# Autodesk Inventor assembly: Eje delantero _1_
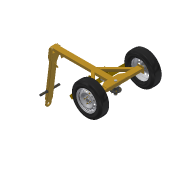
[picture p0: Inventor's stored thumbnail of the model, 180x180]
Saved by Autodesk Inventor 2019 (Build 230136000, 136)
## iProperties
Created: 2020-02-06
Part Number: Eje delantero _1_
Document SubType Name: Assembly
Designer: Juan Carlos Botero
Author: Juan Carlos Botero
## Documents named in this file (26)
- D:\Drives\OneDrive\Carlos_2\02 TRABAJOS\MULTIPLO\Conveyor\ENSAMBLE\Eje delantero _1_.iam
- D:\Drives\OneDrive\Carlos_2\02 TRABAJOS\MULTIPLO\Conveyor\ENSAMBLE\Seguro de tiro.ipt
- D:\Drives\OneDrive\Carlos_2\02 TRABAJOS\MULTIPLO\Conveyor\ENSAMBLE\Lamina bocin rueda.ipt
- D:\Drives\OneDrive\Carlos_2\02 TRABAJOS\MULTIPLO\Conveyor\ENSAMBLE\Lamina refuerzo eje quinta rueda.ipt
- D:\Drives\OneDrive\Carlos_2\02 TRABAJOS\MULTIPLO\Conveyor\ENSAMBLE\Lamina refuerzo tiro.ipt
- D:\Drives\OneDrive\Carlos_2\02 TRABAJOS\MULTIPLO\Conveyor\ENSAMBLE\Perfil tiro.ipt
- D:\Drives\OneDrive\Carlos_2\02 TRABAJOS\MULTIPLO\Conveyor\ENSAMBLE\Espaciador de nylon.ipt
- D:\Drives\OneDrive\Carlos_2\02 TRABAJOS\MULTIPLO\Conveyor\ENSAMBLE\Arandela de nylon (1).ipt
- D:\Drives\OneDrive\Carlos_2\02 TRABAJOS\MULTIPLO\Conveyor\ENSAMBLE\Refuerzo diagonal tiro (1).ipt
- D:\Drives\OneDrive\Carlos_2\02 TRABAJOS\MULTIPLO\Conveyor\ENSAMBLE\Barra quinta rueda.ipt
- D:\Drives\OneDrive\Carlos_2\02 TRABAJOS\MULTIPLO\Conveyor\ENSAMBLE\Lamina pivote seguro tiro.ipt
- D:\Drives\OneDrive\Carlos_2\02 TRABAJOS\MULTIPLO\Conveyor\ENSAMBLE\Tapa perfiles tiro.ipt
- D:\Drives\OneDrive\Carlos_2\02 TRABAJOS\MULTIPLO\Conveyor\ENSAMBLE\Rin 13_.ipt
- D:\Drives\OneDrive\Carlos_2\02 TRABAJOS\MULTIPLO\Conveyor\ENSAMBLE\70 R13.ipt
- D:\Drives\OneDrive\Carlos_2\02 TRABAJOS\MULTIPLO\Conveyor\ENSAMBLE\Bocin llantas _2_.iam
- D:\Drives\OneDrive\Carlos_2\02 TRABAJOS\MULTIPLO\Conveyor\ENSAMBLE\Bocin eje quinta rueda _1_.iam
- D:\Drives\OneDrive\Carlos_2\02 TRABAJOS\MULTIPLO\Conveyor\ENSAMBLE\Bocin llantas _1_.iam
- D:\Drives\OneDrive\Carlos_2\02 TRABAJOS\MULTIPLO\Conveyor\ENSAMBLE\Barra freno.ipt
- D:\Drives\OneDrive\Carlos_2\02 TRABAJOS\MULTIPLO\Conveyor\ENSAMBLE\Soporte freno.ipt
- D:\Drives\OneDrive\Carlos_2\02 TRABAJOS\MULTIPLO\Conveyor\ENSAMBLE\Soporte resorte freno.ipt
- D:\Drives\OneDrive\Carlos_2\02 TRABAJOS\MULTIPLO\Conveyor\ENSAMBLE\Eje delantero _1_\Design Accelerator\Extension Spring2.iam
- D:\Drives\OneDrive\Carlos_2\02 TRABAJOS\MULTIPLO\Conveyor\ENSAMBLE\Solid1.ipt
- D:\Drives\OneDrive\Carlos_2\02 TRABAJOS\MULTIPLO\Conveyor\ENSAMBLE\Barra de freno.ipt
- D:\Drives\OneDrive\Carlos_2\02 TRABAJOS\MULTIPLO\Conveyor\ENSAMBLE\Soporte pivote freno.ipt
- D:\Drives\OneDrive\Carlos_2\02 TRABAJOS\MULTIPLO\Conveyor\ENSAMBLE\Eje de accionamiento freno.ipt
- D:\Drives\OneDrive\Carlos_2\02 TRABAJOS\MULTIPLO\Conveyor\ENSAMBLE\Manillar_freno.iam
## Components (36 placed, 25 different names)
1. Seguro de tiro:1
2. Lamina bocin rueda:1 — Symmetry:1
3. Lamina refuerzo eje quinta rueda:1
4. Lamina refuerzo eje quinta rueda:2 — Mate:5
5. Perfil tiro:1 — Flush:2, Flush:3
6. Espaciador de nylon:11
7. Lamina refuerzo tiro:3
8. Arandela de nylon (1):1
9. Arandela de nylon (1):2
10. Refuerzo diagonal tiro (1):1 — Mate:26
11. Barra quinta rueda:1
12. Lamina pivote seguro tiro:1
13. Refuerzo diagonal tiro (1):2 — Mate:27
14. Lamina pivote seguro tiro:2
15. Tapa perfiles tiro:2
16. Lamina bocin rueda:2 — Symmetry:1
17. Espaciador de nylon:12
18. Rin 13":3
19. 70 R13:3
20. Lamina refuerzo tiro:6
21. 70 R13:4
22. Rin 13":4
23. Bocin llantas <2>:1 [sub-assembly]
24. Bocin eje quinta rueda <1>:1 [sub-assembly]
25. Bocin llantas <1>:1 [sub-assembly]
26. Barra freno:1 — Mate:7, Flush:3, Mate:12, Mate:13, Mate:14, Mate:15, Mate:22, Mate:23
27. Soporte freno:1 — Mate:8, Mate:25
28. Soporte resorte freno:1 — Flush:2, Mate:5, Rotational:3, Mate:6
29. Extension Spring:1 [sub-assembly] — Rotational:3
30. Solid1:1 — Mate:12, Mate:13, Mate:25, Rotational:6
31. Solid1:2 — Mate:14, Mate:15, Mate:18, Angle:1, Rotational:5
32. Barra de freno:1 — Rotational:7
33. Soporte pivote freno:1 — Rotational:5, Mate:26
34. Soporte pivote freno:2 — Rotational:6, Mate:27
35. Eje de accionamiento freno:1 — Mate:22, Mate:23, Rotational:7
36. Manillar_freno:1 [sub-assembly]
## Relationships (25: Mate 14, RevoluteJoint 6, Flush 3, Symmetry 1, Angle 1)
- Flush:2: Perfil tiro:1 ↔ Soporte resorte freno:1
- Symmetry:1: Lamina bocin rueda:1 ↔ Lamina bocin rueda:2
- Mate:5: Lamina refuerzo eje quinta rueda:2 ↔ Soporte resorte freno:1
- Rotational:3 [RevoluteJoint]: Soporte resorte freno:1 ↔ Extension Spring:1
- Mate:6: Soporte resorte freno:1
- Mate:7: Barra freno:1
- Flush:3 (-50 mm): Perfil tiro:1 ↔ Barra freno:1
- Mate:8: Soporte freno:1
- Mate:12: Barra freno:1 ↔ Solid1:1
- Mate:13: Barra freno:1 ↔ Solid1:1
- Mate:14: Barra freno:1 ↔ Solid1:2
- Mate:15: Barra freno:1 ↔ Solid1:2
- [RevoluteJoint]: Espaciador de nylon:12 ↔ Manillar_freno:1
- Mate:18: Solid1:2
- Angle:1 (0 deg): Solid1:2
- Mate:22: Barra freno:1 ↔ Eje de accionamiento freno:1
- Mate:23: Barra freno:1 ↔ Eje de accionamiento freno:1
- [Flush]: Eje de accionamiento freno:1 ↔ Manillar_freno:1
- Rotational:5 [RevoluteJoint]: Solid1:2 ↔ Soporte pivote freno:1
- Mate:25: Soporte freno:1 ↔ Solid1:1
- Mate:26: Refuerzo diagonal tiro (1):1 ↔ Soporte pivote freno:1
- Rotational:6 [RevoluteJoint]: Solid1:1 ↔ Soporte pivote freno:2
- Mate:27: Refuerzo diagonal tiro (1):2 ↔ Soporte pivote freno:2
- Rotational:7 [RevoluteJoint]: Barra de freno:1 ↔ Eje de accionamiento freno:1
- [RevoluteJoint]: Barra de freno:1 ↔ Manillar_freno:1
